# Autodesk Inventor assembly: 42146-27
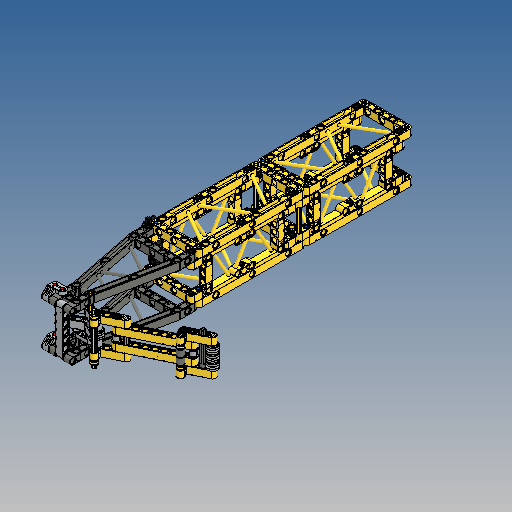
[picture p0: Inventor's stored thumbnail of the model, 512x512]
Saved by Autodesk Inventor 2025 (Build 290162010, 162A)
## iProperties
Created: 2024-12-02
Part Number: 42146-27
Material: Generisch
Document SubType Name: Assembly
Designer: hp.muther
Author: hp.muther
## Documents named in this file (27)
- D:\Inventor\Projekte\Muther\LEGO Technic\LEGO Technik - Raupenkran LR 13000 (42146)\42146-27.iam
- D:\Inventor\Projekte\Muther\LEGO Technic\LEGO Pieces\Rahmen, T-Stücke\79766-Yellow.ipt
- D:\Inventor\Projekte\Muther\LEGO Technic\LEGO Pieces\Pin's\2780-Black.ipt
- D:\Inventor\Projekte\Muther\LEGO Technic\LEGO Pieces\Pin's\43093-Blue.ipt
- D:\Inventor\Projekte\Muther\LEGO Technic\LEGO Pieces\Rahmen, T-Stücke\79767-Yellow.ipt
- D:\Inventor\Projekte\Muther\LEGO Technic\LEGO Pieces\Achsen\44294-Yellow.ipt
- D:\Inventor\Projekte\Muther\LEGO Technic\LEGO Pieces\Achsen\3705-Black.ipt
- D:\Inventor\Projekte\Muther\LEGO Technic\LEGO Pieces\Pin's\3673-LtBluishGray.ipt
- D:\Inventor\Projekte\Muther\LEGO Technic\LEGO Pieces\Rund\18654-DkBluishGray.ipt
- D:\Inventor\Projekte\Muther\LEGO Technic\LEGO Pieces\Rund\4265c-Yellow.ipt
- D:\Inventor\Projekte\Muther\LEGO Technic\LEGO Pieces\Verbindungselemente\41678-Black.ipt
- D:\Inventor\Projekte\Muther\LEGO Technic\LEGO Pieces\Verbindungselemente\63869-Black.ipt
- D:\Inventor\Projekte\Muther\LEGO Technic\LEGO Pieces\Rahmen, T-Stücke\79768-DkBluishGray.ipt
- D:\Inventor\Projekte\Muther\LEGO Technic\LEGO Pieces\Lochbalken\40490-Yellow.ipt
- D:\Inventor\Projekte\Muther\LEGO Technic\LEGO Pieces\Pin's\11214-Red.ipt
- D:\Inventor\Projekte\Muther\LEGO Technic\LEGO Pieces\Pin's\32054-LtBluishGray.ipt
- D:\Inventor\Projekte\Muther\LEGO Technic\LEGO Pieces\Winkel\32140-Yellow.ipt
- D:\Inventor\Projekte\Muther\LEGO Technic\LEGO Pieces\Achsen\32209-DkBluishGray.ipt
- D:\Inventor\Projekte\Muther\LEGO Technic\LEGO Pieces\Achsen\32073-LtBluishGray.ipt
- D:\Inventor\Projekte\Muther\LEGO Technic\LEGO Pieces\Räder, Raupe\42610-LtBluishGray.ipt
- D:\Inventor\Projekte\Muther\LEGO Technic\LEGO Pieces\Winkel\32348-LtBluishGray.ipt
- D:\Inventor\Projekte\Muther\LEGO Technic\LEGO Pieces\Achsen\4519-Yellow.ipt
- D:\Inventor\Projekte\Muther\LEGO Technic\LEGO Pieces\Verbindungselemente\61408-LtBluishGray.ipt
- D:\Inventor\Projekte\Muther\LEGO Technic\LEGO Pieces\Lochbalken\32524-LtBluishGray.ipt
- D:\Inventor\Projekte\Muther\LEGO Technic\LEGO Pieces\Pin's\6558-Blue.ipt
- D:\Inventor\Projekte\Muther\LEGO Technic\LEGO Pieces\Verbindungselemente\92907-LtBluishGray.ipt
- D:\Inventor\Projekte\Muther\LEGO Technic\LEGO Pieces\Achsen\32062-Red.ipt
## Components (96 placed, 26 different names)
1. 79766-Yellow:1 — Einfügen:1, Einfügen:2, Einfügen:3, Einfügen:4, Einfügen:5, Einfügen:6, Einfügen:7, Einfügen:31, Einfügen:32, Einfügen:35
2. 2780-Black:1 — Einfügen:4
3. 2780-Black:2 — Einfügen:6
4. 2780-Black:3 — Einfügen:3
5. 2780-Black:4 — Einfügen:5, Passend:1
6. 43093-Blue:1 — Einfügen:2
7. 43093-Blue:2 — Einfügen:1
8. 2780-Black:5 — Einfügen:31
9. 2780-Black:6 — Einfügen:32, Passend:7
10. 79767-Yellow:1 — Einfügen:7, Passend:1, Einfügen:15, Passend:3
11. 79766-Yellow:2 — Einfügen:14, Einfügen:15, Einfügen:33, Einfügen:34
12. 2780-Black:7
13. 2780-Black:8 — Passend:3
14. 2780-Black:9
15. 2780-Black:10 — Passend:2
16. 43093-Blue:3
17. 43093-Blue:4
18. 79767-Yellow:2 — Einfügen:14, Passend:2
19. 79766-Yellow:3 — Einfügen:16, Einfügen:17, Einfügen:18, Einfügen:19, Einfügen:20, Einfügen:21, Einfügen:30, Einfügen:40, Einfügen:41
20. 2780-Black:11 — Einfügen:19
21. 2780-Black:12 — Einfügen:21
22. 2780-Black:13 — Einfügen:18
23. 2780-Black:14 — Einfügen:20, Passend:6
24. 43093-Blue:5 — Einfügen:17
25. 43093-Blue:6 — Einfügen:16
26. 2780-Black:15 — Einfügen:33
27. 2780-Black:16 — Einfügen:34
28. 79767-Yellow:3 — Einfügen:22, Passend:4, Einfügen:30, Passend:6, Einfügen:36, Einfügen:37, Einfügen:50, Passend:10
29. 79766-Yellow:4 — Einfügen:23, Einfügen:24, Einfügen:25, Einfügen:26, Einfügen:27, Einfügen:28, Einfügen:29, Einfügen:35, Passend:7, Einfügen:22
30. 2780-Black:17 — Einfügen:26
31. 2780-Black:18 — Einfügen:28, Passend:4
32. 2780-Black:19 — Einfügen:25
33. 2780-Black:20 — Einfügen:27, Passend:5
34. 43093-Blue:7 — Einfügen:24
35. 43093-Blue:8 — Einfügen:23
36. 79767-Yellow:4 — Einfügen:29, Passend:5, Einfügen:38, Einfügen:39, Einfügen:51, Einfügen:87
37. 2780-Black:21 — Einfügen:38
38. 2780-Black:22 — Einfügen:39
39. 2780-Black:23 — Einfügen:36, Passend:23
40. 2780-Black:24 — Einfügen:37, Passend:11
41. 44294-Yellow:1 — Einfügen:41
42. 44294-Yellow:2 — Einfügen:40
43. 3705-Black:1 — Einfügen:42, Passend:8, Passend:9
44. 2780-Black:25 — Einfügen:46
45. 2780-Black:26 — Einfügen:45, Passend:10
46. 3673-LtBluishGray:1 — Einfügen:47, Einfügen:48
47. 18654-DkBluishGray:1 — Einfügen:48
48. 18654-DkBluishGray:2 — Einfügen:49
49. 4265c-Yellow:1 — Einfügen:43, Passend:8, Einfügen:44
50. 41678-Black:1 — Einfügen:44, Passend:9, Einfügen:47, Einfügen:49
51. 63869-Black:1 — Einfügen:42, Einfügen:43, Einfügen:45, Einfügen:46, Einfügen:50
52. 79768-DkBluishGray:1 — Einfügen:51, Passend:11, Einfügen:86, Passend:22, Einfügen:88, Einfügen:90, Einfügen:92, Passend:25
53. 40490-Yellow:1 — Einfügen:52, Einfügen:58, Passend:12, Einfügen:71
54. 2780-Black:27 — Einfügen:52
55. 11214-Red:1 — Einfügen:53, Einfügen:57
56. 32054-LtBluishGray:1 — Einfügen:53, Passend:12, Passend:19
57. 32140-Yellow:1 — Einfügen:59, Passend:13, Einfügen:60, Einfügen:61, Einfügen:62, Einfügen:69
58. 40490-Yellow:2 — Einfügen:56, Einfügen:57, Einfügen:72, Passend:16
59. 2780-Black:28 — Einfügen:59
60. 11214-Red:2 — Einfügen:56, Passend:13
61. 32054-LtBluishGray:2 — Einfügen:58, Passend:15
62. 32209-DkBluishGray:1 — Einfügen:60
63. 32073-LtBluishGray:1 — Einfügen:61
64. 42610-LtBluishGray:1 — Einfügen:62, Einfügen:63
65. 42610-LtBluishGray:2 — Einfügen:63, Einfügen:64
66. 42610-LtBluishGray:3 — Einfügen:64
67. 32073-LtBluishGray:2 — Einfügen:66, Passend:14
68. 18654-DkBluishGray:3 — Einfügen:65, Einfügen:68
69. 4265c-Yellow:2 — Einfügen:65, Einfügen:66, Passend:14
70. 18654-DkBluishGray:4 — Einfügen:68
71. 4265c-Yellow:3 — Einfügen:69
72. 32140-Yellow:2 — Einfügen:72, Einfügen:81
73. 32073-LtBluishGray:3 — Passend:16
74. 32140-Yellow:3 — Einfügen:71, Passend:15
75. 32348-LtBluishGray:1 — Einfügen:73, Passend:17, Einfügen:74, Einfügen:75, Einfügen:78, Einfügen:79, Einfügen:81
76. 4519-Yellow:1 — Einfügen:75, Passend:27, Fluchtend:1
77. 32073-LtBluishGray:4 — Einfügen:73, Passend:17, Passend:18
78. 42610-LtBluishGray:4 — Einfügen:74
79. 44294-Yellow:3 — Einfügen:77, Passend:22
80. 18654-DkBluishGray:5 — Einfügen:79
81. 61408-LtBluishGray:1 — Einfügen:77, Einfügen:78, Einfügen:86
82. 32348-LtBluishGray:2 — Passend:18, Einfügen:82, Passend:27, Fluchtend:1, Winkel:1
83. 32140-Yellow:4 — Einfügen:82, Passend:19, Einfügen:85
84. 44294-Yellow:4 — Einfügen:83, Einfügen:84, Passend:20, Passend:21
85. 4265c-Yellow:4 — Einfügen:84, Passend:20, Einfügen:85
86. 4265c-Yellow:5 — Einfügen:83, Passend:21
87. 79768-DkBluishGray:2 — Einfügen:87, Passend:23, Einfügen:89, Einfügen:91, Passend:26
88. 32524-LtBluishGray:1 — Einfügen:90, Passend:24, Winkel:1
89. 6558-Blue:1 — Einfügen:88
90. 6558-Blue:2 — Einfügen:89, Passend:24
91. 92907-LtBluishGray:1 — Einfügen:91, Passend:26, Einfügen:93, Einfügen:95
92. 92907-LtBluishGray:2 — Einfügen:92, Passend:25, Einfügen:94, Einfügen:96
93. 32062-Red:1 — Einfügen:93
94. 32062-Red:2 — Einfügen:94
95. 32062-Red:3 — Einfügen:96
96. 32062-Red:4 — Einfügen:95
## Relationships (123: Insert 94, Mate 27, Flush 1, Angle 1)
- Einfügen:1 [Insert]: 79766-Yellow:1 ↔ 43093-Blue:2
- Einfügen:2 [Insert]: 79766-Yellow:1 ↔ 43093-Blue:1
- Einfügen:3 [Insert]: 79766-Yellow:1 ↔ 2780-Black:3
- Einfügen:4 [Insert]: 79766-Yellow:1 ↔ 2780-Black:1
- Einfügen:5 [Insert]: 79766-Yellow:1 ↔ 2780-Black:4
- Einfügen:6 [Insert]: 79766-Yellow:1 ↔ 2780-Black:2
- Einfügen:7 [Insert]: 79766-Yellow:1 ↔ 79767-Yellow:1
- Passend:1 [Mate]: 2780-Black:4 ↔ 79767-Yellow:1
- [Insert]: 79766-Yellow:2 ↔ 43093-Blue:4
- [Insert]: 79766-Yellow:2 ↔ 43093-Blue:3
- [Insert]: 79766-Yellow:2 ↔ 2780-Black:9
- [Insert]: 79766-Yellow:2 ↔ 2780-Black:7
- [Insert]: 79766-Yellow:2 ↔ 2780-Black:10
- [Insert]: 79766-Yellow:2 ↔ 2780-Black:8
- Einfügen:14 [Insert]: 79766-Yellow:2 ↔ 79767-Yellow:2
- Passend:2 [Mate]: 2780-Black:10 ↔ 79767-Yellow:2
- Einfügen:15 [Insert]: 79767-Yellow:1 ↔ 79766-Yellow:2
- Passend:3 [Mate]: 79767-Yellow:1 ↔ 2780-Black:8
- Einfügen:16 [Insert]: 79766-Yellow:3 ↔ 43093-Blue:6
- Einfügen:17 [Insert]: 79766-Yellow:3 ↔ 43093-Blue:5
- Einfügen:18 [Insert]: 79766-Yellow:3 ↔ 2780-Black:13
- Einfügen:19 [Insert]: 79766-Yellow:3 ↔ 2780-Black:11
- Einfügen:20 [Insert]: 79766-Yellow:3 ↔ 2780-Black:14
- Einfügen:21 [Insert]: 79766-Yellow:3 ↔ 2780-Black:12
- Einfügen:22 [Insert]: 79767-Yellow:3 ↔ 79766-Yellow:4
- Passend:4 [Mate]: 79767-Yellow:3 ↔ 2780-Black:18
- Einfügen:23 [Insert]: 79766-Yellow:4 ↔ 43093-Blue:8
- Einfügen:24 [Insert]: 79766-Yellow:4 ↔ 43093-Blue:7
- Einfügen:25 [Insert]: 79766-Yellow:4 ↔ 2780-Black:19
- Einfügen:26 [Insert]: 79766-Yellow:4 ↔ 2780-Black:17
- Einfügen:27 [Insert]: 79766-Yellow:4 ↔ 2780-Black:20
- Einfügen:28 [Insert]: 79766-Yellow:4 ↔ 2780-Black:18
- Einfügen:29 [Insert]: 79766-Yellow:4 ↔ 79767-Yellow:4
- Passend:5 [Mate]: 2780-Black:20 ↔ 79767-Yellow:4
- Einfügen:30 [Insert]: 79766-Yellow:3 ↔ 79767-Yellow:3
- Passend:6 [Mate]: 2780-Black:14 ↔ 79767-Yellow:3
- Einfügen:31 [Insert]: 79766-Yellow:1 ↔ 2780-Black:5
- Einfügen:32 [Insert]: 79766-Yellow:1 ↔ 2780-Black:6
- Einfügen:33 [Insert]: 79766-Yellow:2 ↔ 2780-Black:15
- Einfügen:34 [Insert]: 79766-Yellow:2 ↔ 2780-Black:16
- Einfügen:35 [Insert]: 79766-Yellow:1 ↔ 79766-Yellow:4
- Passend:7 [Mate]: 2780-Black:6 ↔ 79766-Yellow:4
- Einfügen:36 [Insert]: 79767-Yellow:3 ↔ 2780-Black:23
- Einfügen:37 [Insert]: 79767-Yellow:3 ↔ 2780-Black:24
- Einfügen:38 [Insert]: 79767-Yellow:4 ↔ 2780-Black:21
- Einfügen:39 [Insert]: 79767-Yellow:4 ↔ 2780-Black:22
- Einfügen:40 [Insert]: 79766-Yellow:3 ↔ 44294-Yellow:2
- Einfügen:41 [Insert]: 79766-Yellow:3 ↔ 44294-Yellow:1
- Einfügen:42 [Insert]: 3705-Black:1 ↔ 63869-Black:1
- Einfügen:43 [Insert]: 4265c-Yellow:1 ↔ 63869-Black:1
- Passend:8 [Mate]: 3705-Black:1 ↔ 4265c-Yellow:1
- Einfügen:44 [Insert]: 4265c-Yellow:1 ↔ 41678-Black:1
- Passend:9 [Mate]: 3705-Black:1 ↔ 41678-Black:1
- Einfügen:45 [Insert]: 2780-Black:26 ↔ 63869-Black:1
- Einfügen:46 [Insert]: 2780-Black:25 ↔ 63869-Black:1
- Einfügen:47 [Insert]: 3673-LtBluishGray:1 ↔ 41678-Black:1
- Einfügen:48 [Insert]: 3673-LtBluishGray:1 ↔ 18654-DkBluishGray:1
- Einfügen:49 [Insert]: 18654-DkBluishGray:2 ↔ 41678-Black:1
- Einfügen:50 [Insert]: 79767-Yellow:3 ↔ 63869-Black:1
- Passend:10 [Mate]: 79767-Yellow:3 ↔ 2780-Black:26
- Einfügen:51 [Insert]: 79767-Yellow:4 ↔ 79768-DkBluishGray:1
- Passend:11 [Mate]: 2780-Black:24 ↔ 79768-DkBluishGray:1
- Einfügen:52 [Insert]: 40490-Yellow:1 ↔ 2780-Black:27
- Einfügen:53 [Insert]: 11214-Red:1 ↔ 32054-LtBluishGray:1
- [Insert]: 40490-Yellow:2 ↔ 2780-Black:28
- [Insert]: 11214-Red:2 ↔ 32054-LtBluishGray:2
- Einfügen:56 [Insert]: 40490-Yellow:2 ↔ 11214-Red:2
- Einfügen:57 [Insert]: 11214-Red:1 ↔ 40490-Yellow:2
- Einfügen:58 [Insert]: 40490-Yellow:1 ↔ 32054-LtBluishGray:2
- Passend:12 [Mate]: 40490-Yellow:1 ↔ 32054-LtBluishGray:1
- Einfügen:59 [Insert]: 32140-Yellow:1 ↔ 2780-Black:28
- Passend:13 [Mate]: 32140-Yellow:1 ↔ 11214-Red:2
- Einfügen:60 [Insert]: 32140-Yellow:1 ↔ 32209-DkBluishGray:1
- Einfügen:61 [Insert]: 32140-Yellow:1 ↔ 32073-LtBluishGray:1
- Einfügen:62 [Insert]: 32140-Yellow:1 ↔ 42610-LtBluishGray:1
- Einfügen:63 [Insert]: 42610-LtBluishGray:1 ↔ 42610-LtBluishGray:2
- Einfügen:64 [Insert]: 42610-LtBluishGray:2 ↔ 42610-LtBluishGray:3
- Einfügen:65 [Insert]: 18654-DkBluishGray:3 ↔ 4265c-Yellow:2
- Einfügen:66 [Insert] (-12 mm): 32073-LtBluishGray:2 ↔ 4265c-Yellow:2
- Passend:14 [Mate]: 32073-LtBluishGray:2 ↔ 4265c-Yellow:2
- [Insert]: 18654-DkBluishGray:4 ↔ 4265c-Yellow:3
- Einfügen:68 [Insert]: 18654-DkBluishGray:3 ↔ 18654-DkBluishGray:4
- Einfügen:69 [Insert]: 32140-Yellow:1 ↔ 4265c-Yellow:3
- [Insert]: 32140-Yellow:2 ↔ 32073-LtBluishGray:3
- Einfügen:71 [Insert]: 40490-Yellow:1 ↔ 32140-Yellow:3
- Passend:15 [Mate]: 32054-LtBluishGray:2 ↔ 32140-Yellow:3
- Einfügen:72 [Insert]: 40490-Yellow:2 ↔ 32140-Yellow:2
- Passend:16 [Mate]: 40490-Yellow:2 ↔ 32073-LtBluishGray:3
- Einfügen:73 [Insert] (-16 mm): 32348-LtBluishGray:1 ↔ 32073-LtBluishGray:4
- Passend:17 [Mate]: 32348-LtBluishGray:1 ↔ 32073-LtBluishGray:4
- Einfügen:74 [Insert]: 32348-LtBluishGray:1 ↔ 42610-LtBluishGray:4
- Einfügen:75 [Insert] (-8 mm): 32348-LtBluishGray:1 ↔ 4519-Yellow:1
- Einfügen:77 [Insert] (-16 mm): 44294-Yellow:3 ↔ 61408-LtBluishGray:1
- Einfügen:78 [Insert]: 32348-LtBluishGray:1 ↔ 61408-LtBluishGray:1
- Einfügen:79 [Insert]: 32348-LtBluishGray:1 ↔ 18654-DkBluishGray:5
- Passend:18 [Mate]: 32073-LtBluishGray:4 ↔ 32348-LtBluishGray:2
- Einfügen:81 [Insert]: 32140-Yellow:2 ↔ 32348-LtBluishGray:1
- Einfügen:82 [Insert]: 32348-LtBluishGray:2 ↔ 32140-Yellow:4
- Passend:19 [Mate]: 32054-LtBluishGray:1 ↔ 32140-Yellow:4
- Einfügen:83 [Insert] (-8 mm): 44294-Yellow:4 ↔ 4265c-Yellow:5
- Einfügen:84 [Insert] (-8 mm): 44294-Yellow:4 ↔ 4265c-Yellow:4
- Passend:20 [Mate]: 44294-Yellow:4 ↔ 4265c-Yellow:4
- Passend:21 [Mate]: 44294-Yellow:4 ↔ 4265c-Yellow:5
- Einfügen:85 [Insert]: 32140-Yellow:4 ↔ 4265c-Yellow:4
- Einfügen:86 [Insert]: 79768-DkBluishGray:1 ↔ 61408-LtBluishGray:1
- Passend:22 [Mate]: 79768-DkBluishGray:1 ↔ 44294-Yellow:3
- Einfügen:87 [Insert]: 79767-Yellow:4 ↔ 79768-DkBluishGray:2
- Passend:23 [Mate]: 2780-Black:23 ↔ 79768-DkBluishGray:2
- Einfügen:88 [Insert]: 79768-DkBluishGray:1 ↔ 6558-Blue:1
- Einfügen:89 [Insert]: 79768-DkBluishGray:2 ↔ 6558-Blue:2
- Einfügen:90 [Insert]: 79768-DkBluishGray:1 ↔ 32524-LtBluishGray:1
- Passend:24 [Mate]: 32524-LtBluishGray:1 ↔ 6558-Blue:2
- Einfügen:91 [Insert]: 79768-DkBluishGray:2 ↔ 92907-LtBluishGray:1
- Einfügen:92 [Insert]: 79768-DkBluishGray:1 ↔ 92907-LtBluishGray:2
- Passend:25 [Mate]: 79768-DkBluishGray:1 ↔ 92907-LtBluishGray:2
- Passend:26 [Mate]: 79768-DkBluishGray:2 ↔ 92907-LtBluishGray:1
- Einfügen:93 [Insert]: 92907-LtBluishGray:1 ↔ 32062-Red:1
- Einfügen:94 [Insert]: 92907-LtBluishGray:2 ↔ 32062-Red:2
- Einfügen:95 [Insert] (-16 mm): 92907-LtBluishGray:1 ↔ 32062-Red:4
- Einfügen:96 [Insert] (-16 mm): 92907-LtBluishGray:2 ↔ 32062-Red:3
- Passend:27 [Mate]: 4519-Yellow:1 ↔ 32348-LtBluishGray:2
- Fluchtend:1 [Flush]: 4519-Yellow:1 ↔ 32348-LtBluishGray:2
- Winkel:1 [Angle] (26.565 deg): 32348-LtBluishGray:2 ↔ 32524-LtBluishGray:1
## Named parameters: d8_d0 = 0 mm, d9_d1 = 0 mm, d10_d2 = 0 mm, d11_d3 = 0 mm, d12_d4 = 0 mm, d13_d5 = 0 mm, d14_d6 = 0 mm, d15_d7 = 0 mm, d18_d0 = 0 mm, d19_d1 = 0 mm, d20_d2 = 0 mm, d21_d3 = 0 mm, d22_d4 = 0 mm, d23_d5 = 0 mm, d24_d6 = 0 mm, d25_d7 = 0 mm, d26_d8_d0 = 0 mm, d27_d9_d1 = 0 mm, d28_d10_d2 = 0 mm, d29_d11_d3 = 0 mm, d30_d12_d4 = 0 mm, d31_d13_d5 = 0 mm, d32_d14_d6 = 0 mm, d33_d15_d7 = 0 mm, d34_d16 = 0 mm, d35_d17 = 0 mm, d64_d62 = 0 mm, d65_d63 = 0 mm, d80_d77 = 0 mm, d83_d73 = 0 mm
